# Autodesk Inventor assembly: LF_2
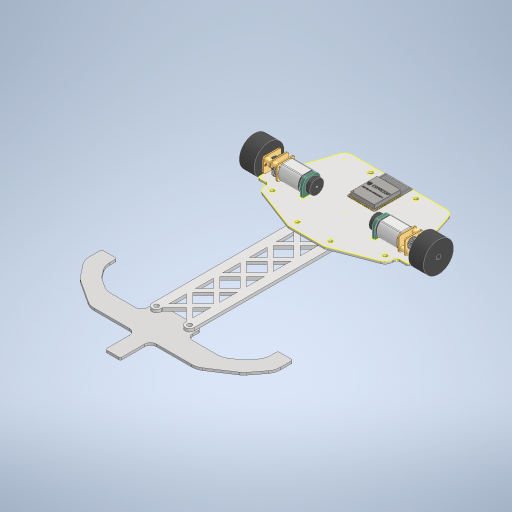
[picture p0: Inventor's stored thumbnail of the model, 512x512]
Saved by Autodesk Inventor 2023 (Build 270158000, 158)
## iProperties
Created: 2024-03-30
Part Number: LF_2
Document SubType Name: Assembly
Designer: Kamil
Author: Kamil
## Documents named in this file (8)
- C:\Users\kamil\Documents\PROJECTS - repos\Line_Follower_ZACZ\mechanics\LF_2.iam
- C:\Users\kamil\Documents\PROJECTS - repos\Line_Follower_ZACZ\mechanics\N20 Mini Micro Metall Gear Motor DC 3-6-12V v1.ipt
- C:\Users\kamil\Documents\PROJECTS - repos\Line_Follower_ZACZ\mechanics\ESP32-S3-WROOM-1.ipt
- C:\Users\kamil\Documents\PROJECTS - repos\Line_Follower_ZACZ\mechanics\przód.ipt
- C:\Users\kamil\Documents\PROJECTS - repos\Line_Follower_ZACZ\mechanics\kolko.ipt
- C:\Users\kamil\Documents\PROJECTS - repos\ModBot---Projekt-Zespolowy\mechanics\N20_Bracket_Extended_Pololu.ipt
- C:\Users\kamil\Documents\PROJECTS - repos\Line_Follower_ZACZ\mechanics\lacznik.ipt
- C:\Users\kamil\Documents\PROJECTS - repos\Line_Follower_ZACZ\mechanics\plytka_glowna.ipt
## Components (10 placed, 7 different names)
1. N20 Mini Micro Metall Gear Motor DC 3-6-12V v1:1 — Zestawiające:27, Zestawiające:28, Zestawiające:29, Równoległe:1, Równoległe:2
2. N20 Mini Micro Metall Gear Motor DC 3-6-12V v1:2 — Zestawiające:30, Zestawiające:31, Zestawiające:32, Równoległe:3, Równoległe:4
3. ESP32-S3-WROOM-1:1 — Zestawiające:39, Równoległe:5, Równoległe:6
4. kolko:1 — Zestawiające:30, Zestawiające:31
5. kolko:2 — Zestawiające:28, Zestawiające:29
6. N20_Bracket_Extended_Pololu:1 — Zestawiające:27, Równoległe:1, Równoległe:2, Zestawiające:33, Zestawiające:37, Zestawiające:38
7. N20_Bracket_Extended_Pololu:2 — Zestawiające:32, Równoległe:3, Równoległe:4, Zestawiające:34, Zestawiające:35, Zestawiające:36
8. przód:1 — Zestawiające:21, Zestawiające:22, Zestawiające:23
9. lacznik:1 — Zestawiające:21, Zestawiające:22, Zestawiające:23, Zestawiające:24, Zestawiające:25, Zestawiające:26
10. plytka_glowna:1 — Zestawiające:24, Zestawiające:25, Zestawiające:26, Zestawiające:33, Zestawiające:34, Zestawiające:35, Zestawiające:36, Zestawiające:37, Zestawiające:38, Zestawiające:39, Równoległe:5, Równoległe:6
## Relationships (25: Mate 19, Flush 6)
- Zestawiające:21 [Mate]: przód:1 ↔ lacznik:1
- Zestawiające:22 [Mate]: przód:1 ↔ lacznik:1
- Zestawiające:23 [Mate]: przód:1 ↔ lacznik:1
- Zestawiające:24 [Mate]: lacznik:1 ↔ plytka_glowna:1
- Zestawiające:25 [Mate]: lacznik:1 ↔ plytka_glowna:1
- Zestawiające:26 [Mate]: lacznik:1 ↔ plytka_glowna:1
- Zestawiające:27 [Mate]: N20 Mini Micro Metall Gear Motor DC 3-6-12V v1:1 ↔ N20_Bracket_Extended_Pololu:1
- Zestawiające:28 [Mate]: N20 Mini Micro Metall Gear Motor DC 3-6-12V v1:1 ↔ kolko:2
- Zestawiające:29 [Mate] (0.5 mm): N20 Mini Micro Metall Gear Motor DC 3-6-12V v1:1 ↔ kolko:2
- Równoległe:1 [Flush]: N20 Mini Micro Metall Gear Motor DC 3-6-12V v1:1 ↔ N20_Bracket_Extended_Pololu:1
- Równoległe:2 [Flush]: N20 Mini Micro Metall Gear Motor DC 3-6-12V v1:1 ↔ N20_Bracket_Extended_Pololu:1
- Zestawiające:30 [Mate] (0.5 mm): N20 Mini Micro Metall Gear Motor DC 3-6-12V v1:2 ↔ kolko:1
- Zestawiające:31 [Mate]: N20 Mini Micro Metall Gear Motor DC 3-6-12V v1:2 ↔ kolko:1
- Zestawiające:32 [Mate]: N20 Mini Micro Metall Gear Motor DC 3-6-12V v1:2 ↔ N20_Bracket_Extended_Pololu:2
- Równoległe:3 [Flush]: N20 Mini Micro Metall Gear Motor DC 3-6-12V v1:2 ↔ N20_Bracket_Extended_Pololu:2
- Równoległe:4 [Flush]: N20 Mini Micro Metall Gear Motor DC 3-6-12V v1:2 ↔ N20_Bracket_Extended_Pololu:2
- Zestawiające:33 [Mate]: N20_Bracket_Extended_Pololu:1 ↔ plytka_glowna:1
- Zestawiające:34 [Mate]: N20_Bracket_Extended_Pololu:2 ↔ plytka_glowna:1
- Zestawiające:35 [Mate]: N20_Bracket_Extended_Pololu:2 ↔ plytka_glowna:1
- Zestawiające:36 [Mate]: N20_Bracket_Extended_Pololu:2 ↔ plytka_glowna:1
- Zestawiające:37 [Mate]: N20_Bracket_Extended_Pololu:1 ↔ plytka_glowna:1
- Zestawiające:38 [Mate]: N20_Bracket_Extended_Pololu:1 ↔ plytka_glowna:1
- Zestawiające:39 [Mate]: ESP32-S3-WROOM-1:1 ↔ plytka_glowna:1
- Równoległe:5 [Flush]: ESP32-S3-WROOM-1:1 ↔ plytka_glowna:1
- Równoległe:6 [Flush] (40.9 mm): ESP32-S3-WROOM-1:1 ↔ plytka_glowna:1
